# Autodesk Inventor assembly: entrance-mesh-assembly
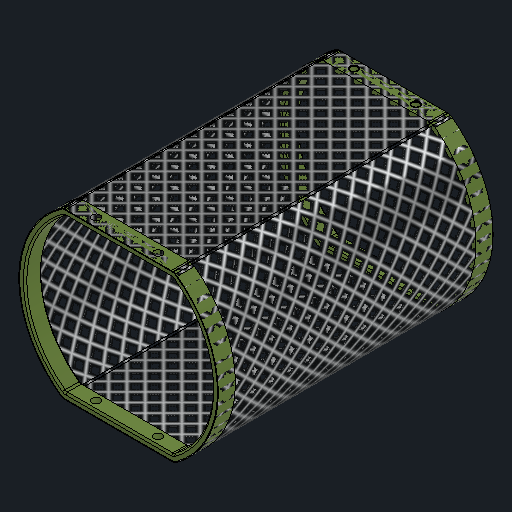
[picture p0: Inventor's stored thumbnail of the model, 512x512]
Saved by Autodesk Inventor 2026 (Build 300175050, 175E)
## iProperties
Created: 2024-05-22
Part Number: entrance-mesh-assembly
Document SubType Name: Assembly
Designer: kuzmin
Author: kuzmin
## Documents named in this file (3)
- C:\Users\queez\Dropbox\Drawings\PIHTI\Plasma Vessel\entrance-mesh-assembly.iam
- C:\Users\queez\Dropbox\Drawings\PIHTI\Plasma Vessel\Plasma-Box\probe-side-large-mesh.ipt
- C:\Users\queez\Dropbox\Drawings\PIHTI\Plasma Vessel\Plasma-Box\plasma-box-probe-window-mesh-holder.ipt
## Components (3 placed, 2 different names)
1. probe-side-large-mesh:1 — Rigid:4, Rigid:3
2. plasma-box-probe-window-mesh-holder:1 — Rigid:4
3. plasma-box-probe-window-mesh-holder:2 — Rigid:3
## Relationships (2: WeldJoint 2)
- Rigid:4 [WeldJoint]: probe-side-large-mesh:1 ↔ plasma-box-probe-window-mesh-holder:1
- Rigid:3 [WeldJoint]: probe-side-large-mesh:1 ↔ plasma-box-probe-window-mesh-holder:2
